# Autodesk Inventor assembly: collector arm wheel1
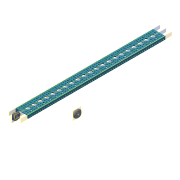
[picture p0: Inventor's stored thumbnail of the model, 180x180]
Saved by Autodesk Inventor 2018 (Build 220112000, 112)
## iProperties
Created: 2018-11-25
Part Number: collector arm wheel1
Document SubType Name: Assembly
Designer: ball
Author: ball
## Documents named in this file (3)
- C:\FTC\FTC8863CAD\2018Robot\collector arm wheel1.iam
- C:\FTC\FTC8863CAD\GoBilda\3600 Parts\3600-0006-2910 Assembly.ipt
- C:\FTC\FTC8863CAD\GoBilda\1121 Parts\1121-0021-0528.ipt
## Components (3 placed, 2 different names)
1. 3600-0006-2910 Assembly:1 — Flush:1
2. 3600-0006-2910 Assembly:2
3. 1121-0021-0528:1 — Flush:1
## Relationships (1: Flush 1)
- Flush:1: 3600-0006-2910 Assembly:1 ↔ 1121-0021-0528:1
